# Autodesk Inventor assembly: HBLTBBN45_MIR_MIR
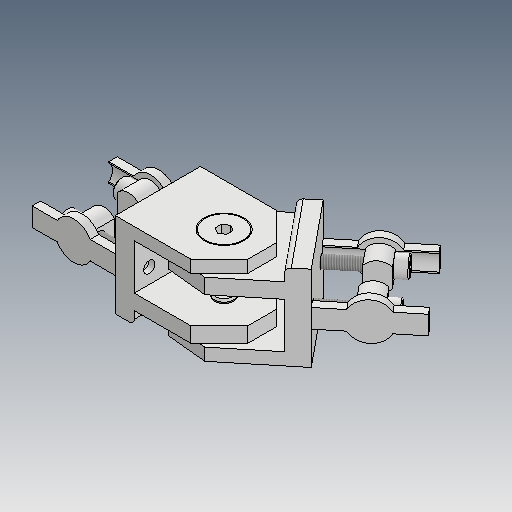
[picture p0: Inventor's stored thumbnail of the model, 512x512]
Saved by Autodesk Inventor 2020 (Build 240168000, 168)
## iProperties
Created: 2021-12-05
Part Number: HBLTBBN45_MIR_MIR
Document SubType Name: Assembly
Designer: magnarecta
Author: ken113
## Documents named in this file (2)
- D:\Documents\GitHub\Eto_Project\Hardware\Parts\MISUMI\HBLTBBN45-SET_Autodesk_Inventor_2020_20211206\AIS2020\HBLTBBN45_MIR_MIR.iam
- D:\Documents\GitHub\Eto_Project\Hardware\Parts\MISUMI\HBLTBBN45-SET_Autodesk_Inventor_2020_20211206\AIS2020\HBLTBBN45-SET_MIR_MIR.iam
## Components (2 placed, 1 different names)
1. HBLTBBN45-SET_MIR_MIR:1 [sub-assembly] — 挿入:1
2. HBLTBBN45-SET_MIR_MIR:2 [sub-assembly] — 挿入:1
## Relationships (1: Insert 1)
- 挿入:1 [Insert]: HBLTBBN45-SET_MIR_MIR:1 ↔ HBLTBBN45-SET_MIR_MIR:2
